# Autodesk Inventor assembly: assy_lower_plates
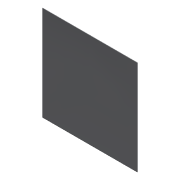
[picture p0: Inventor's stored thumbnail of the model, 180x180]
Saved by Autodesk Inventor 2018 (Build 220112000, 112)
## iProperties
Created: 2017-11-13
Part Number: assy_lower_plates
Document SubType Name: Assembly
Designer: Platform
Author: Platform
## Documents named in this file (2)
- C:\Users\Platform\Desktop\autorace_track\track_model\autorace_rbizchallenge2017\assembled\assy_lower_plates.iam
- C:\Users\Platform\Desktop\RBizChallenge2017_TurtleBot3_AutoRace_map\lower_plate v1.ipt
## Components (4 placed, 1 different names)
1. lower_plate v1:1 — Mate:1, Flush:1, Flush:2, Mate:2, Flush:3, Flush:4
2. lower_plate v1:2 — Mate:1, Flush:1, Flush:2, Mate:3, Flush:5
3. lower_plate v1:3 — Mate:2, Flush:3, Flush:4, Mate:4
4. lower_plate v1:4 — Mate:3, Mate:4, Flush:5
## Relationships (9: Flush 5, Mate 4)
- Mate:1: lower_plate v1:1 ↔ lower_plate v1:2
- Flush:1: lower_plate v1:1 ↔ lower_plate v1:2
- Flush:2: lower_plate v1:1 ↔ lower_plate v1:2
- Mate:2: lower_plate v1:1 ↔ lower_plate v1:3
- Flush:3: lower_plate v1:1 ↔ lower_plate v1:3
- Flush:4: lower_plate v1:1 ↔ lower_plate v1:3
- Mate:3: lower_plate v1:2 ↔ lower_plate v1:4
- Mate:4: lower_plate v1:3 ↔ lower_plate v1:4
- Flush:5: lower_plate v1:2 ↔ lower_plate v1:4
